# Autodesk Inventor assembly: BedAssembly
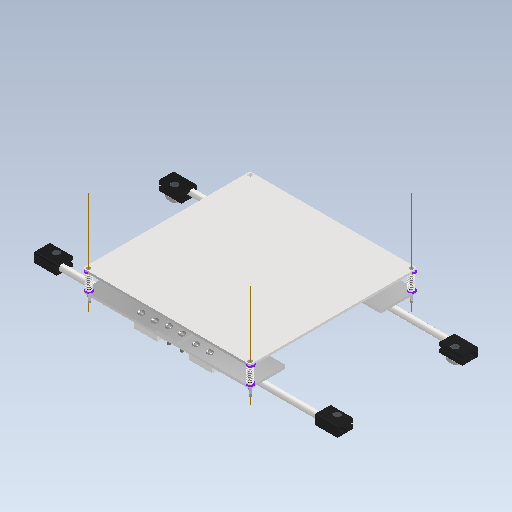
[picture p0: Inventor's stored thumbnail of the model, 512x512]
Saved by Autodesk Inventor 2020.2 (Build 242310000, 310)
## iProperties
Created: 2020-08-19
Part Number: BedAssembly
Document SubType Name: Assembly
Designer: JK
Author: JK
## Documents named in this file (14)
- C:\Users\JK\Documents\Inventor\Anet Upgrade\BedAssembly.iam
- C:\Users\JK\Documents\Inventor\Anet Upgrade\BedCarriageA.ipt
- C:\Users\JK\Documents\Inventor\Anet Upgrade\BedCarriageB.ipt
- C:\Users\JK\Documents\Inventor\Anet Upgrade\Y Belt Attachment A.ipt
- C:\Users\JK\Documents\Inventor\Anet Upgrade\Y Belt Attachment B.ipt
- C:\Users\JK\Documents\Inventor\Anet Upgrade\Bed.ipt
- C:\Users\JK\Documents\Inventor\Anet Upgrade\bedboltassembly.iam
- C:\Users\JK\Documents\Inventor\Anet Upgrade\Bearingandbolts.iam
- C:\Users\JK\Documents\Inventor\Anet Upgrade\M4x20.ipt
- C:\Users\JK\Documents\Inventor\Anet Upgrade\8x380axis.ipt
- C:\Users\JK\Documents\Inventor\Anet Upgrade\YsupportB.ipt
- C:\Users\JK\Documents\Inventor\Anet Upgrade\YsupportA.ipt
- C:\Users\JK\Documents\Inventor\Anet Upgrade\M5x15BoltFlatHead.ipt
- C:\Users\JK\Documents\Inventor\Anet Upgrade\T_Slot_Nut_Dropin_3030m5ipt.ipt
## Components (36 placed, 13 different names)
1. BedCarriageA:1 — Mate:1, Mate:2, Mate:10, Mate:13, Mate:14, Mate:15, Mate:43
2. BedCarriageB:1 — Mate:1, Mate:2, Mate:3, Flush:2, Mate:4, Mate:22, Mate:23, Mate:24, Mate:25, Mate:26, Mate:27, Mate:28
3. Y Belt Attachment A:1 — Mate:3, Flush:2, Mate:4, Mate:5, Flush:3, Mate:6
4. Y Belt Attachment B:1 — Mate:5, Flush:3, Mate:6, Mate:16, Mate:17, Mate:18, Mate:19, Mate:20, Mate:21
5. Bed:1 — Mate:11, Mate:12, Flush:5, Flush:6, Flush:7
6. bedboltassembly:2 [sub-assembly] — Mate:12, Flush:5, Mate:43
7. bedboltassembly:3 [sub-assembly] — Mate:10, Flush:6
8. bedboltassembly:4 [sub-assembly] — Mate:11, Flush:7
9. AS 1427 Z - Metryczny M4 x 20:1 — Mate:17, Flush:8, Mate:20
10. AS 1427 Z - Metryczny M4 x 20:2 — Mate:16, Flush:9
11. AS 1427 Z - Metryczny M4 x 20:3 — Mate:18, Flush:9, Mate:21
12. AS 1427 Z - Metryczny M4 x 20:4 — Mate:19, Flush:8
13. AS 1427 Z - Metryczny M4 x 20:5 — Mate:22, Flush:12, Flush:13
14. AS 1427 Z - Metryczny M4 x 20:6 — Mate:23, Flush:13, Flush:14
15. AS 1427 Z - Metryczny M4 x 20:7 — Mate:27, Flush:10, Flush:11
16. AS 1427 Z - Metryczny M4 x 20:8 — Mate:25, Flush:11, Flush:12
17. AS 1427 Z - Metryczny M4 x 20:9 — Mate:26, Flush:10
18. AS 1427 Z - Metryczny M4 x 20:10 — Mate:24, Flush:14, Mate:28
19. Wał:1 — Mate:29, Flush:15, Mate:33, Mate:35, Mate:36
20. Wał:2 — Mate:30, Flush:15, Mate:32, Mate:34, Mate:37
21. YsupportB:1 — Mate:35, Flush:19, Flush:20, Mate:36, Mate:40, Angle:2
22. YsupportB:2 — Mate:32, Flush:16, Flush:17, Flush:18, Mate:37, Mate:38, Mate:42, Angle:4
23. YsupportA:1 — Mate:33, Flush:16, Flush:18, Mate:39, Angle:3
24. YsupportA:2 — Mate:34, Flush:17, Flush:19, Flush:20, Mate:41, Angle:1, Mate:48
25. M5x15BoltFlatHead:1 — Mate:38, Flush:23, Mate:42, Mate:46
26. M5x15BoltFlatHead:2 — Mate:39, Flush:22, Flush:23, Mate:45
27. M5x15BoltFlatHead:3 — Mate:41, Flush:21, Mate:47
28. M5x15BoltFlatHead:4 — Mate:40, Flush:21, Flush:22, Mate:44
29. T_Slot_Nut_Dropin_3030m5ipt:1 — Mate:44, Flush:26, Angle:2
30. T_Slot_Nut_Dropin_3030m5ipt:2 — Mate:45, Flush:24, Angle:3
31. T_Slot_Nut_Dropin_3030m5ipt:3 — Mate:46, Flush:24, Flush:25, Angle:4
32. T_Slot_Nut_Dropin_3030m5ipt:4 — Mate:47, Flush:25, Flush:26, Angle:1, Mate:48
33. Bearingandbolts:1 [sub-assembly] — Mate:13, Mate:14, Mate:15
34. Bearingandbolts:2 [sub-assembly]
35. Bearingandbolts:3 [sub-assembly] — Mate:30
36. Bearingandbolts:4 [sub-assembly] — Mate:29
## Component patterns: (4 elements, first: Bearingandbolts:1)
## Relationships (72: Mate 44, Flush 24, Angle 4)
- Mate:1: BedCarriageA:1 ↔ BedCarriageB:1
- Mate:2: BedCarriageA:1 ↔ BedCarriageB:1
- Mate:3: BedCarriageB:1 ↔ Y Belt Attachment A:1
- Flush:2: BedCarriageB:1 ↔ Y Belt Attachment A:1
- Mate:4: BedCarriageB:1 ↔ Y Belt Attachment A:1
- Mate:5: Y Belt Attachment A:1 ↔ Y Belt Attachment B:1
- Flush:3: Y Belt Attachment A:1 ↔ Y Belt Attachment B:1
- Mate:6 (1.6 mm): Y Belt Attachment A:1 ↔ Y Belt Attachment B:1
- Mate:10: BedCarriageA:1 ↔ bedboltassembly:3
- Mate:11: Bed:1 ↔ bedboltassembly:4
- Mate:12: Bed:1 ↔ bedboltassembly:2
- Flush:5: Bed:1 ↔ bedboltassembly:2
- Flush:6: Bed:1 ↔ bedboltassembly:3
- Flush:7: Bed:1 ↔ bedboltassembly:4
- Mate:13: BedCarriageA:1 ↔ Bearingandbolts:1
- Mate:14: BedCarriageA:1 ↔ Bearingandbolts:1
- Mate:15: BedCarriageA:1 ↔ Bearingandbolts:1
- Mate:16: Y Belt Attachment B:1 ↔ AS 1427 Z - Metryczny M4 x 20:2
- Mate:17: Y Belt Attachment B:1 ↔ AS 1427 Z - Metryczny M4 x 20:1
- Mate:18: Y Belt Attachment B:1 ↔ AS 1427 Z - Metryczny M4 x 20:3
- Mate:19: Y Belt Attachment B:1 ↔ AS 1427 Z - Metryczny M4 x 20:4
- Flush:8: AS 1427 Z - Metryczny M4 x 20:1 ↔ AS 1427 Z - Metryczny M4 x 20:4
- Flush:9: AS 1427 Z - Metryczny M4 x 20:2 ↔ AS 1427 Z - Metryczny M4 x 20:3
- Mate:20: Y Belt Attachment B:1 ↔ AS 1427 Z - Metryczny M4 x 20:1
- Mate:21: Y Belt Attachment B:1 ↔ AS 1427 Z - Metryczny M4 x 20:3
- Mate:22: BedCarriageB:1 ↔ AS 1427 Z - Metryczny M4 x 20:5
- Mate:23: BedCarriageB:1 ↔ AS 1427 Z - Metryczny M4 x 20:6
- Mate:24: BedCarriageB:1 ↔ AS 1427 Z - Metryczny M4 x 20:10
- Mate:25: BedCarriageB:1 ↔ AS 1427 Z - Metryczny M4 x 20:8
- Mate:26: BedCarriageB:1 ↔ AS 1427 Z - Metryczny M4 x 20:9
- Mate:27: BedCarriageB:1 ↔ AS 1427 Z - Metryczny M4 x 20:7
- Flush:10: AS 1427 Z - Metryczny M4 x 20:7 ↔ AS 1427 Z - Metryczny M4 x 20:9
- Flush:11: AS 1427 Z - Metryczny M4 x 20:7 ↔ AS 1427 Z - Metryczny M4 x 20:8
- Flush:12: AS 1427 Z - Metryczny M4 x 20:5 ↔ AS 1427 Z - Metryczny M4 x 20:8
- Flush:13: AS 1427 Z - Metryczny M4 x 20:5 ↔ AS 1427 Z - Metryczny M4 x 20:6
- Flush:14: AS 1427 Z - Metryczny M4 x 20:6 ↔ AS 1427 Z - Metryczny M4 x 20:10
- Mate:28: BedCarriageB:1 ↔ AS 1427 Z - Metryczny M4 x 20:10
- Mate:29: Wał:1 ↔ Bearingandbolts:4
- Mate:30: Wał:2 ↔ Bearingandbolts:3
- Flush:15: Wał:1 ↔ Wał:2
- Mate:32: Wał:2 ↔ YsupportB:2
- Mate:33: Wał:1 ↔ YsupportA:1
- Flush:16: YsupportB:2 ↔ YsupportA:1
- Mate:34: Wał:2 ↔ YsupportA:2
- Flush:17: YsupportB:2 ↔ YsupportA:2
- Flush:18: YsupportB:2 ↔ YsupportA:1
- Mate:35: Wał:1 ↔ YsupportB:1
- Flush:19: YsupportB:1 ↔ YsupportA:2
- Flush:20: YsupportB:1 ↔ YsupportA:2
- Mate:36: Wał:1 ↔ YsupportB:1
- Mate:37: Wał:2 ↔ YsupportB:2
- Mate:38: YsupportB:2 ↔ M5x15BoltFlatHead:1
- Mate:39: YsupportA:1 ↔ M5x15BoltFlatHead:2
- Mate:40: YsupportB:1 ↔ M5x15BoltFlatHead:4
- Mate:41: YsupportA:2 ↔ M5x15BoltFlatHead:3
- Flush:21: M5x15BoltFlatHead:3 ↔ M5x15BoltFlatHead:4
- Flush:22: M5x15BoltFlatHead:2 ↔ M5x15BoltFlatHead:4
- Flush:23: M5x15BoltFlatHead:1 ↔ M5x15BoltFlatHead:2
- Mate:42: YsupportB:2 ↔ M5x15BoltFlatHead:1
- Mate:43: BedCarriageA:1 ↔ bedboltassembly:2
- Mate:44: M5x15BoltFlatHead:4 ↔ T_Slot_Nut_Dropin_3030m5ipt:1
- Mate:45: M5x15BoltFlatHead:2 ↔ T_Slot_Nut_Dropin_3030m5ipt:2
- Mate:46: M5x15BoltFlatHead:1 ↔ T_Slot_Nut_Dropin_3030m5ipt:3
- Mate:47: M5x15BoltFlatHead:3 ↔ T_Slot_Nut_Dropin_3030m5ipt:4
- Flush:24: T_Slot_Nut_Dropin_3030m5ipt:2 ↔ T_Slot_Nut_Dropin_3030m5ipt:3
- Flush:25: T_Slot_Nut_Dropin_3030m5ipt:3 ↔ T_Slot_Nut_Dropin_3030m5ipt:4
- Flush:26: T_Slot_Nut_Dropin_3030m5ipt:1 ↔ T_Slot_Nut_Dropin_3030m5ipt:4
- Angle:1 (90 deg): YsupportA:2 ↔ T_Slot_Nut_Dropin_3030m5ipt:4
- Mate:48: YsupportA:2 ↔ T_Slot_Nut_Dropin_3030m5ipt:4
- Angle:2 (0 deg): YsupportB:1 ↔ T_Slot_Nut_Dropin_3030m5ipt:1
- Angle:3 (0 deg): YsupportA:1 ↔ T_Slot_Nut_Dropin_3030m5ipt:2
- Angle:4 (0 deg): YsupportB:2 ↔ T_Slot_Nut_Dropin_3030m5ipt:3
